# Autodesk Inventor assembly: Robot
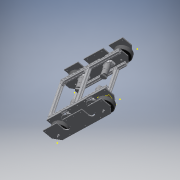
[picture p0: Inventor's stored thumbnail of the model, 180x180]
Saved by Autodesk Inventor 2016 (Build 200138000, 138)
## iProperties
Created: 2016-10-08
Part Number: Robot
Document SubType Name: Assembly
Designer: RoboticsUser
Author: RoboticsUser
## Documents named in this file (7)
- C:\Robotics\2016-17_CAD\Robot.iam
- C:\Robotics\2016-17_CAD\WheelAssemblyWFrame.iam
- C:\Robotics\CAD\2015-16\COTSParts\Bosch Extrusion\Bosch 20x20 9 in.ipt
- C:\Robotics\CAD\2015-16\COTSParts\Bosch Extrusion\Gusset 20x20 w screws.ipt
- C:\Robotics\CAD\2015-16\COTSParts\Bosch Extrusion\Bosch 20x20 9 in - Copy.ipt
- C:\Robotics\CAD\2015-16\COTSParts\Bosch Extrusion\Rexroth-6mmT-Nutm4.ipt
- C:\Robotics\CAD\2015-16\COTSParts\Bosch Extrusion\Rexroth-GussetwFastenersm4x8.ipt
## Components (23 placed, 6 different names)
1. WheelAssemblyWFrame:1 [sub-assembly] — Mate:1, Insert:4, Insert:5, Insert:6, Flush:29, Mate:55, Flush:36, Flush:37
2. WheelAssemblyWFrame:2 [sub-assembly] — Mate:8, Mate:9, Flush:7, Flush:8, Insert:1, Insert:2, Insert:3, Flush:30, Flush:35, Mate:57, Mate:58
3. Bosch 20x20 9 in:1 — Flush:36, Flush:37, Mate:56, Mate:58
4. Gusset 20x20 w screws:1 — Mate:9, Flush:7, Mate:10
5. Gusset 20x20 w screws:2 — Mate:1
6. Gusset 20x20 w screws:3 — Mate:8
7. Gusset 20x20 w screws:4 — Mate:11, Flush:9
8. Bosch 20x20 9 in:2 — Mate:10, Flush:8, Mate:11, Flush:9, Flush:35, Mate:55
9. Bosch 20x20 9 in - Copy:1 — Mate:33, Flush:25, Flush:28, Flush:30, Flush:31, Mate:44, Flush:34, Mate:52, Mate:53
10. Rexroth-6mmT-Nutm4:1 — Insert:1
11. Rexroth-6mmT-Nutm4:2 — Insert:3, Mate:33, Flush:25
12. Rexroth-6mmT-Nutm4:3 — Insert:2
13. Bosch 20x20 9 in - Copy:2 — Mate:15, Flush:11, Mate:35, Mate:39, Flush:27, Flush:29, Flush:32, Mate:48, Flush:33, Mate:54
14. Rexroth-6mmT-Nutm4:4 — Insert:4
15. Rexroth-6mmT-Nutm4:5 — Insert:5
16. Rexroth-6mmT-Nutm4:6 — Insert:6, Mate:15, Flush:11
17. Bosch 20x20 9 in:3 — Flush:27, Flush:31, Mate:50, Mate:51, Mate:53, Mate:54
18. Bosch 20x20 9 in:4 — Mate:39, Flush:28, Flush:32, Mate:45, Mate:46, Mate:47, Mate:49, Flush:33, Flush:34
19. Gusset 20x20 w screws:5 — Mate:51, Mate:52
20. Gusset 20x20 w screws:6 — Mate:35, Mate:50
21. Gusset 20x20 w screws:7 — Mate:47, Mate:48, Mate:49
22. Gusset 20x20 w screws:8 — Mate:44, Mate:45, Mate:46
23. Rexroth-GussetwFastenersm4x8:4 — Mate:56, Mate:57
## Relationships (46: Mate 24, Flush 16, Insert 6)
- Mate:1: WheelAssemblyWFrame:1 ↔ Gusset 20x20 w screws:2
- Mate:8: WheelAssemblyWFrame:2 ↔ Gusset 20x20 w screws:3
- Mate:9: WheelAssemblyWFrame:2 ↔ Gusset 20x20 w screws:1
- Flush:7: WheelAssemblyWFrame:2 ↔ Gusset 20x20 w screws:1
- Mate:10: Gusset 20x20 w screws:1 ↔ Bosch 20x20 9 in:2
- Flush:8: WheelAssemblyWFrame:2 ↔ Bosch 20x20 9 in:2
- Mate:11: Gusset 20x20 w screws:4 ↔ Bosch 20x20 9 in:2
- Flush:9: Gusset 20x20 w screws:4 ↔ Bosch 20x20 9 in:2
- Insert:1: WheelAssemblyWFrame:2 ↔ Rexroth-6mmT-Nutm4:1
- Insert:2: WheelAssemblyWFrame:2 ↔ Rexroth-6mmT-Nutm4:3
- Insert:3: WheelAssemblyWFrame:2 ↔ Rexroth-6mmT-Nutm4:2
- Insert:4: WheelAssemblyWFrame:1 ↔ Rexroth-6mmT-Nutm4:4
- Insert:5: WheelAssemblyWFrame:1 ↔ Rexroth-6mmT-Nutm4:5
- Insert:6: WheelAssemblyWFrame:1 ↔ Rexroth-6mmT-Nutm4:6
- Mate:15: Bosch 20x20 9 in - Copy:2 ↔ Rexroth-6mmT-Nutm4:6
- Flush:11 (64.77 mm): Bosch 20x20 9 in - Copy:2 ↔ Rexroth-6mmT-Nutm4:6
- Mate:33: Bosch 20x20 9 in - Copy:1 ↔ Rexroth-6mmT-Nutm4:2
- Flush:25 (64.77 mm): Bosch 20x20 9 in - Copy:1 ↔ Rexroth-6mmT-Nutm4:2
- Mate:35: Bosch 20x20 9 in - Copy:2 ↔ Gusset 20x20 w screws:6
- Mate:39: Bosch 20x20 9 in - Copy:2 ↔ Bosch 20x20 9 in:4
- Flush:27: Bosch 20x20 9 in - Copy:2 ↔ Bosch 20x20 9 in:3
- Flush:28: Bosch 20x20 9 in - Copy:1 ↔ Bosch 20x20 9 in:4
- Flush:29 (1.6256 mm): WheelAssemblyWFrame:1 ↔ Bosch 20x20 9 in - Copy:2
- Flush:30 (1.6256 mm): WheelAssemblyWFrame:2 ↔ Bosch 20x20 9 in - Copy:1
- Flush:31 (56.896 mm): Bosch 20x20 9 in - Copy:1 ↔ Bosch 20x20 9 in:3
- Flush:32: Bosch 20x20 9 in - Copy:2 ↔ Bosch 20x20 9 in:4
- Mate:44: Bosch 20x20 9 in - Copy:1 ↔ Gusset 20x20 w screws:8
- Mate:45: Bosch 20x20 9 in:4 ↔ Gusset 20x20 w screws:8
- Mate:46: Bosch 20x20 9 in:4 ↔ Gusset 20x20 w screws:8
- Mate:47: Bosch 20x20 9 in:4 ↔ Gusset 20x20 w screws:7
- Mate:48: Bosch 20x20 9 in - Copy:2 ↔ Gusset 20x20 w screws:7
- Mate:49: Bosch 20x20 9 in:4 ↔ Gusset 20x20 w screws:7
- Flush:33: Bosch 20x20 9 in - Copy:2 ↔ Bosch 20x20 9 in:4
- Flush:34: Bosch 20x20 9 in - Copy:1 ↔ Bosch 20x20 9 in:4
- Mate:50: Bosch 20x20 9 in:3 ↔ Gusset 20x20 w screws:6
- Mate:51: Bosch 20x20 9 in:3 ↔ Gusset 20x20 w screws:5
- Mate:52: Bosch 20x20 9 in - Copy:1 ↔ Gusset 20x20 w screws:5
- Mate:53: Bosch 20x20 9 in - Copy:1 ↔ Bosch 20x20 9 in:3
- Mate:54: Bosch 20x20 9 in - Copy:2 ↔ Bosch 20x20 9 in:3
- Flush:35 (218.6178 mm): WheelAssemblyWFrame:2 ↔ Bosch 20x20 9 in:2
- Mate:55: WheelAssemblyWFrame:1 ↔ Bosch 20x20 9 in:2
- Flush:36: WheelAssemblyWFrame:1 ↔ Bosch 20x20 9 in:1
- Flush:37: WheelAssemblyWFrame:1 ↔ Bosch 20x20 9 in:1
- Mate:56: Bosch 20x20 9 in:1 ↔ Rexroth-GussetwFastenersm4x8:4
- Mate:57: WheelAssemblyWFrame:2 ↔ Rexroth-GussetwFastenersm4x8:4
- Mate:58: WheelAssemblyWFrame:2 ↔ Bosch 20x20 9 in:1
